# Autodesk Inventor assembly: Montagem1
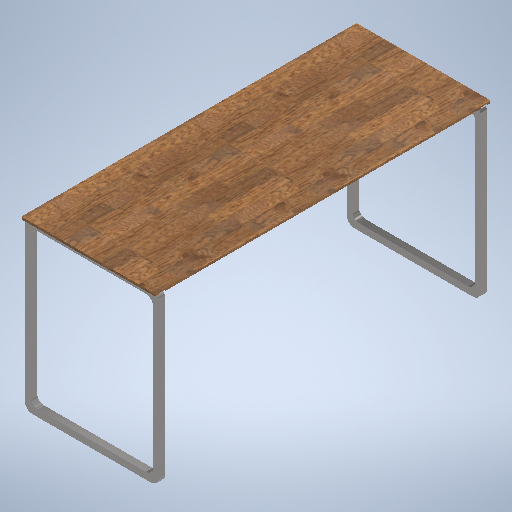
[picture p0: Inventor's stored thumbnail of the model, 512x512]
Saved by Autodesk Inventor 2025.2 (Build 292293000, 293)
## iProperties
Created: 2025-04-02
Part Number: Montagem1
Document SubType Name: Assembly
Designer: kenay
Author: kenay
## Documents named in this file (3)
- C:\Users\kenay\Downloads\Mesa Ergonômica\Montagem1.iam
- C:\Users\kenay\Downloads\Mesa Ergonômica\Pés.ipt
- C:\Users\kenay\Downloads\Mesa Ergonômica\Superfície.ipt
## Components (3 placed, 2 different names)
1. Superfície:1 — Alinhado:1, Alinhado:2, Alinhado:3, Alinhado:4, Alinhado:5, Alinhado:6, Alinhado:7, Coincidente:5
2. Pés:1 — Alinhado:6, Alinhado:8, Coincidente:4, Simetria:1
3. Pés:2 — Alinhado:8, Coincidente:4, Simetria:1, Alinhado:7, Coincidente:5
## Relationships (11: Flush 8, Mate 2, Symmetry 1)
- Alinhado:1 [Flush]: Superfície:1
- Alinhado:2 [Flush]: Superfície:1
- Alinhado:3 [Flush]: Superfície:1
- Alinhado:4 [Flush]: Superfície:1
- Alinhado:5 [Flush]: Superfície:1
- Alinhado:6 [Flush]: Superfície:1 ↔ Pés:1
- Alinhado:8 [Flush]: Pés:1 ↔ Pés:2
- Coincidente:4 [Mate]: Pés:1 ↔ Pés:2
- Simetria:1 [Symmetry]: Pés:1 ↔ Pés:2
- Alinhado:7 [Flush] (15 mm): Superfície:1 ↔ Pés:2
- Coincidente:5 [Mate]: Superfície:1 ↔ Pés:2
